# Autodesk Inventor assembly: Cooling Fan, 40mm x 40mm x 10 mm, 12VDC
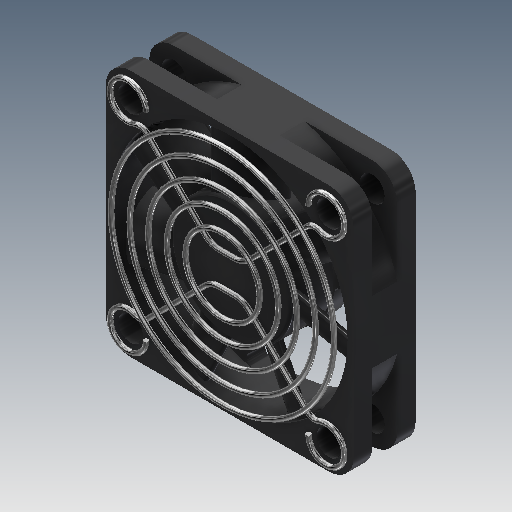
[picture p0: Inventor's stored thumbnail of the model, 512x512]
Saved by Autodesk Inventor 2019.1 (Build 231200000, 200)
## iProperties
Created: 2005-12-01
Part Number: Cooling Fan, 40mm x 40mm x 10 mm, 12VDC
Document SubType Name: Assembly
Designer: floress
Mass: 7.15013 g
Surface Area: 82.7702 cm^2
Volume: 7.15013 cm^3
Density: 1 g/cm^3
Author: floress
## Documents named in this file (3)
- C:\Vault Workspace\Process Equipment\Workspace\Supplier Content\Electrical Design\Motherboard\Processor Fan\Cooling Fan, 40mm x 40mm x 10 mm, 12VDC.iam
- C:\Vault Workspace\Process Equipment\Workspace\Supplier Content\Electrical Design\Motherboard\Processor Fan\Cooling Fan, 40mm x 40mm x 10 mm, 12VDC.ipt
- C:\Vault Workspace\Process Equipment\Workspace\Supplier Content\Electrical Design\Motherboard\Processor Fan\Fan Guard, 40mm.ipt
## Components (2 placed, 2 different names)
1. Cooling Fan, 40mm x 40mm x 10 mm, 12VDC:1 — Mate:2, Mate:3, Tangent:1
2. Fan Guard, 40mm:1 — Mate:2, Mate:3, Tangent:1
## Relationships (3: Mate 2, Tangent 1)
- Mate:2: Cooling Fan, 40mm x 40mm x 10 mm, 12VDC:1 ↔ Fan Guard, 40mm:1
- Mate:3: Cooling Fan, 40mm x 40mm x 10 mm, 12VDC:1 ↔ Fan Guard, 40mm:1
- Tangent:1: Cooling Fan, 40mm x 40mm x 10 mm, 12VDC:1 ↔ Fan Guard, 40mm:1
